# Autodesk Inventor assembly: SCSW12-10
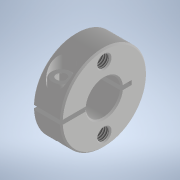
[picture p0: Inventor's stored thumbnail of the model, 180x180]
Saved by Autodesk Inventor 2021 (Build 250183000, 183)
## iProperties
Category: PARTsolutions
Company: MISUMI
Created: 2025-01-13
Part Number: SCSW12-10
Catalog Web Link: www.cadenas.de
Description: SCSW, PSCSW, SSCSW, SCSWA, SCSWAW-Set Collars - Slit 2 Hole/2 Tap - Standard Type - 2 Tap Type
Vendor: MISUMI
Document SubType Name: Assembly
Designer: psAdmin
Manufacturer: MISUMI
Mass: 5.31223 g
Surface Area: 33.6403 cm^2
Volume: 5.31223 cm^3
Density: 1 g/cm^3
Title: SCSW12-10
Author: Cadenas PARTsolutions
Comments: Set Collars - Slit 2 Hole/2 Tap - Standard Type - 2 Tap Type
PSOL_IDENT_0: {$CADENAS_DATA/23d-libs/misumi/metric/03_set_collars/scsw_asmtab.prj},210 {VTYP=3D},{STYP=ASSTAB},{N
PSOL_IDENT_1: B=SCSW12-10},{LINA=SCSW12-10},{NN=SCSW, PSCSW, SSCSW, SCSWA, SCSWAW},{DATE=29.11.2024 04:05:21},{GEO
PSOL_IDENT_2: MDATE=15.09.2021 06:02:54},{VERSION=},{LINEID=70},{WBVAR=MAT,ST,BS},{WBNUMERIC=BS}  {NB=SCSW12-10},{
PSOL_IDENT_3: LINA=SCSW12-10},{KT=DUMMY},{PN=SCSW12-10},{TYPE=SCSW},{MAT=1045},{MATA='1045','S45C Equivalent','304'
PSOL_IDENT_4: ,'SUS304 Equivalent','2017','2017 Aluminum Alloy'},{ST=Black Oxide},{AC=Hexagon Socket Head Set Scre
PSOL_IDENT_5: w 1 Pc.},{D=12},{BS=10},{B1=8,10,12,15},{D1=30},{M=M4},{THMD=4},{THDMIN=3.242},{ST0='Black Oxide','B
PSOL_IDENT_6: lack Oxide','Electroless Nickel Plating','Electroless Nickel Plating'},{DD=4.5},{R=3.75},{W=1.5},{X=
PSOL_IDENT_7: 10.0},{Y=5.0},{Z=9~10},{S=5.5},{P=22},{C=0.5},{L=12},{M1=M5},{ZZ=9.5},{THMD1=5},{THDMIN1=4.134},{PPA
PSOL_IDENT_8: TH=scsw_templ.prj}
NB: SCSW12-10
NN: SCSW, PSCSW, SSCSW, SCSWA, SCSWAW
NT: Set Collars - Slit 2 Hole/2 Tap - Standard Type - 2 Tap Type
NBSYN: $PN.
LINA: SCSW12-10
CATALOG: Misumi
PN: SCSW12-10
MAT: S45C Equivalent
ST: Black Oxide
AC: Hexagon Socket Head Set Screw 1 Pc.
D: 12
BS: 10
D1: 30
M: M4
DD: 4.5
R: 3.75
W: 1.5
X: 10
Y: 5
Z: 9~10
S: 5.5
P: 22
M1: M5
SUPPLIER: MISUMI
ARTICLENO: SCSW12-10
BOMINFO: SCSW12-10
CREATOR: CADENAS GmbH
## Documents named in this file (3)
- e:\temp\worker_COMMON_119\temp\tmp_1684_10_VrvzF\format_0\SCSW12-10.iam
- e:\temp\worker_COMMON_119\temp\tmp_1684_10_VrvzF\format_0\SCSW12-10b.ipt
- e:\temp\worker_COMMON_119\temp\tmp_1684_10_VrvzF\format_0\Slotted head cap screw ISO 4762 - M4x12.ipt
## Components (2 placed, 2 different names)
1. SCSW12-10b:1 — body_screw_Z@1 <-> IP1_Z@2
2. Slotted head cap screw ISO 4762 - M4x12:1 — body_screw_Z@1 <-> IP1_Z@2
## Relationships (1: Mate 1)
- body_screw_Z@1 <-> IP1_Z@2 [Mate]: SCSW12-10b:1 ↔ Slotted head cap screw ISO 4762 - M4x12:1
